# Autodesk Inventor assembly: писюны
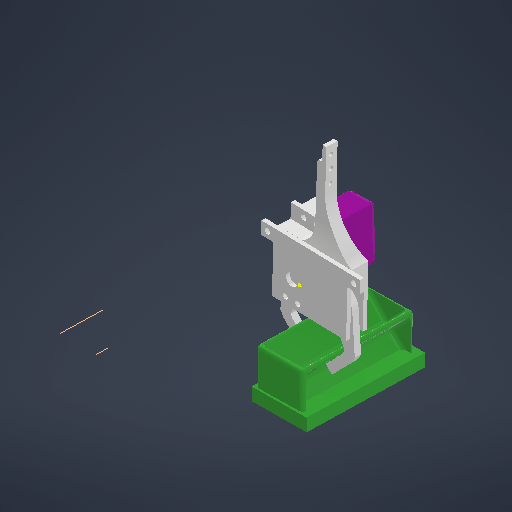
[picture p0: Inventor's stored thumbnail of the model, 512x512]
Saved by Autodesk Inventor 2025 (Build 290162000, 162)
## iProperties
Created: 2024-12-28
Part Number: писюны
Document SubType Name: Assembly
Designer: Phantom
Author: Phantom
## Documents named in this file (8)
- C:\Users\GameHD\Desktop\phantom 16950\писюны.iam
- C:\Users\GameHD\Desktop\phantom 16950\писюн.ipt
- C:\Users\GameHD\Desktop\phantom 16950\писюн 2.ipt
- C:\Users\GameHD\Desktop\phantom 16950\держать писюны.ipt
- C:\Users\GameHD\Desktop\phantom 16950\am-5401 Sample_MIR1.ipt
- C:\Users\GameHD\Desktop\phantom 16950\2000-0025-0002\2000-0025-0002_MIR4.ipt
- C:\Users\GameHD\Downloads\Telegram Desktop\tetrix_metal_servo_horn\tetrix_metal_servo_horn.ipt
- C:\Users\GameHD\Desktop\phantom 16950\держать писюны 2ч.ipt
## Components (7 placed, 7 different names)
1. am-5401 Sample_MIR1:1 — Совмещение:23, Совмещение:24
2. 2000-0025-0002_MIR4:1 — Совмещение:10, Совмещение:11, Совмещение:17
3. tetrix_metal_servo_horn:1 — Совмещение:10, Совмещение:11, Совмещение:15, Совмещение:16, Совмещение:18, Совмещение:19
4. держать писюны:1 — Совмещение:16, Совмещение:17, Совмещение:22, Заподлицо:1
5. писюн 2:1 — Совмещение:18, Совмещение:24
6. писюн:1 — Совмещение:15, Совмещение:19, Совмещение:21, Совмещение:23
7. держать писюны 2ч:1 — Совмещение:21, Совмещение:22, Заподлицо:1
## Relationships (12: Mate 11, Flush 1)
- Совмещение:10 [Mate]: 2000-0025-0002_MIR4:1 ↔ tetrix_metal_servo_horn:1
- Совмещение:11 [Mate]: 2000-0025-0002_MIR4:1 ↔ tetrix_metal_servo_horn:1
- Совмещение:15 [Mate]: tetrix_metal_servo_horn:1 ↔ писюн:1
- Совмещение:16 [Mate]: tetrix_metal_servo_horn:1 ↔ держать писюны:1
- Совмещение:17 [Mate]: 2000-0025-0002_MIR4:1 ↔ держать писюны:1
- Совмещение:18 [Mate]: tetrix_metal_servo_horn:1 ↔ писюн 2:1
- Совмещение:19 [Mate]: tetrix_metal_servo_horn:1 ↔ писюн:1
- Совмещение:21 [Mate]: писюн:1 ↔ держать писюны 2ч:1
- Совмещение:22 [Mate]: держать писюны:1 ↔ держать писюны 2ч:1
- Заподлицо:1 [Flush]: держать писюны:1 ↔ держать писюны 2ч:1
- Совмещение:23 [Mate]: am-5401 Sample_MIR1:1 ↔ писюн:1
- Совмещение:24 [Mate]: am-5401 Sample_MIR1:1 ↔ писюн 2:1
